# Autodesk Inventor assembly: wheel1_MIR
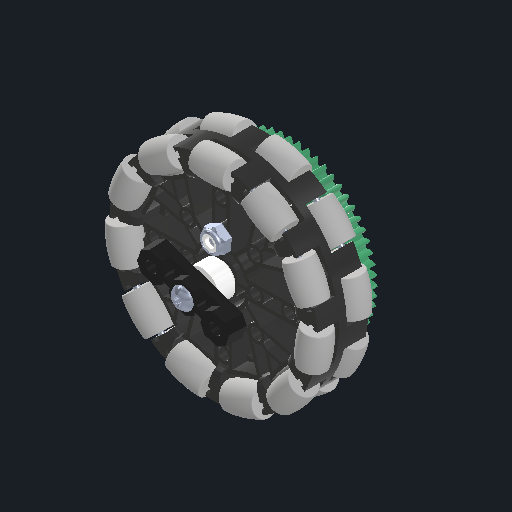
[picture p0: Inventor's stored thumbnail of the model, 512x512]
Saved by Autodesk Inventor 2024 (Build 280153000, 153)
## iProperties
Created: 2023-08-09
Part Number: wheel1_MIR
Document SubType Name: Assembly
Designer: macbook
Author: macbook
## Documents named in this file (15)
- \\Mac\Home\Desktop\code\7899V-VRC-OVER-UNDER\Cad\VEX-CAD-Inventor-1.4.0\Assembly\v0.2\wheel1_MIR.iam
- \\Mac\Home\Desktop\code\7899V-VRC-OVER-UNDER\Cad\VEX-CAD-Inventor-1.4.0\Motion\Gears\LS 60T Gear_MIR.ipt
- \\Mac\Home\Desktop\code\7899V-VRC-OVER-UNDER\Cad\VEX-CAD-Inventor-1.4.0\Motion\Wheels\Omni Wheel\3.25 Omni AS, Circle_MIR.iam
- \\Mac\Home\Desktop\code\7899V-VRC-OVER-UNDER\Cad\VEX-CAD-Inventor-1.4.0\Motion\Spacers\Spacer Nylon .500 OD\NSpacer White .500 OD x .125.ipt
- \\Mac\Home\Desktop\code\7899V-VRC-OVER-UNDER\Cad\VEX-CAD-Inventor-1.4.0\Motion\Spacers\Spacer Nylon .500 OD.ipt
- \\Mac\Home\Desktop\code\7899V-VRC-OVER-UNDER\Cad\VEX-CAD-Inventor-1.4.0\Motion\Spacers\Spacer Nylon .500 OD\NSpacer White .500 OD x .250.ipt
- \\Mac\Home\Desktop\code\7899V-VRC-OVER-UNDER\Cad\VEX-CAD-Inventor-1.4.0\Motion\Spacers\Washer Teflon\TWasher .375 OD x .03125.ipt
- \\Mac\Home\Desktop\code\7899V-VRC-OVER-UNDER\Cad\VEX-CAD-Inventor-1.4.0\Motion\Spacers\Washer Teflon.ipt
- \\Mac\Home\Desktop\code\7899V-VRC-OVER-UNDER\Cad\VEX-CAD-Inventor-1.4.0\Motion\Shaft LS\Bearing Flat_MIR1.ipt
- \\Mac\Home\Desktop\code\7899V-VRC-OVER-UNDER\Cad\VEX-CAD-Inventor-1.4.0\Structure\Hardware\Screw Steel - Star\SScrew Star Smooth 2.250.ipt
- \\Mac\Home\Desktop\code\7899V-VRC-OVER-UNDER\Cad\VEX-CAD-Inventor-1.4.0\Structure\Hardware\Screw Steel - Star.ipt
- \\Mac\Home\Desktop\code\7899V-VRC-OVER-UNDER\Cad\VEX-CAD-Inventor-1.4.0\Motion\Spacers\Spacer Nylon .500 OD\NSpacer White .500 OD x .375.ipt
- \\Mac\Home\Desktop\code\7899V-VRC-OVER-UNDER\Cad\VEX-CAD-Inventor-1.4.0\Structure\Hardware\Screw Steel - Star\SScrew Star Smooth 1.000.ipt
- \\Mac\Home\Desktop\code\7899V-VRC-OVER-UNDER\Cad\VEX-CAD-Inventor-1.4.0\Structure\Hardware\Nut Thin Nylock_MIR1.ipt
- \\Mac\Home\Desktop\code\7899V-VRC-OVER-UNDER\Cad\VEX-CAD-Inventor-1.4.0\Structure\Hardware\Nut Nylock_MIR1.ipt
## Components (16 placed, 11 different names)
1. LS 60T Gear_MIR:1 — Insert:24, Insert:25, Insert:26, Insert:29, Insert:10, Insert:31
2. 3.25 Omni AS, Circle_MIR:1 [sub-assembly]
3. NSpacer White .500 OD x .125:1 — Insert:30
4. NSpacer White .500 OD x .250:2
5. TWasher .375 OD x .03125:1 — Insert:36, Insert:10
6. Bearing Flat_MIR1:1 — Insert:41, Insert:17, Insert:16
7. Bearing Flat_MIR1:2 — Insert:41, Insert:17, Insert:36, Insert:42
8. SScrew Star Smooth 2.250:1 — Insert:16
9. NSpacer White .500 OD x .375:3 — Insert:24
10. NSpacer White .500 OD x .375:4 — Insert:25
11. SScrew Star Smooth 1.000:2 — Insert:26
12. Nut Thin Nylock_MIR1:1
13. Nut Thin Nylock_MIR1:2
14. SScrew Star Smooth 1.000:3 — Insert:29
15. TWasher .375 OD x .03125:2 — Insert:31, Insert:30
16. Nut Nylock_MIR1:1 — Insert:42
## Relationships (12: Insert 12)
- Insert:41 (38.1 mm): Bearing Flat_MIR1:1 ↔ Bearing Flat_MIR1:2
- Insert:17 (38.1 mm): Bearing Flat_MIR1:1 ↔ Bearing Flat_MIR1:2
- Insert:16: Bearing Flat_MIR1:1 ↔ SScrew Star Smooth 2.250:1
- Insert:24: LS 60T Gear_MIR:1 ↔ NSpacer White .500 OD x .375:3
- Insert:25: LS 60T Gear_MIR:1 ↔ NSpacer White .500 OD x .375:4
- Insert:26: LS 60T Gear_MIR:1 ↔ SScrew Star Smooth 1.000:2
- Insert:29: LS 60T Gear_MIR:1 ↔ SScrew Star Smooth 1.000:3
- Insert:36 (1.5875 mm): TWasher .375 OD x .03125:1 ↔ Bearing Flat_MIR1:2
- Insert:10: LS 60T Gear_MIR:1 ↔ TWasher .375 OD x .03125:1
- Insert:31: LS 60T Gear_MIR:1 ↔ TWasher .375 OD x .03125:2
- Insert:30: NSpacer White .500 OD x .125:1 ↔ TWasher .375 OD x .03125:2
- Insert:42: Bearing Flat_MIR1:2 ↔ Nut Nylock_MIR1:1
